# Autodesk Inventor assembly: Battery_Pack
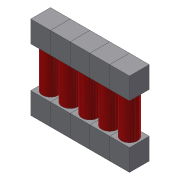
[picture p0: Inventor's stored thumbnail of the model, 180x180]
Saved by Autodesk Inventor 2018 (Build 220112000, 112)
## iProperties
Created: 2019-09-04
Part Number: Battery_Pack
Document SubType Name: Assembly
Designer: Clevo
Author: Clevo
## Documents named in this file (2)
- E:\Hardware_Accelerated_Robot\Hardware\Battery\Battery_Pack.iam
- E:\Hardware_Accelerated_Robot\Hardware\Battery\Battery_Module.iam
## Components (5 placed, 1 different names)
1. Battery_Module:1 [sub-assembly] — Mate:1, Flush:1, Flush:2, Mate:2, Flush:3, Flush:4
2. Battery_Module:2 [sub-assembly] — Mate:1, Flush:1, Flush:2, Mate:4, Flush:7, Flush:8
3. Battery_Module:3 [sub-assembly] — Mate:2, Flush:3, Flush:4, Mate:3, Flush:5, Flush:6
4. Battery_Module:4 [sub-assembly] — Mate:3, Flush:5, Flush:6
5. Battery_Module:5 [sub-assembly] — Mate:4, Flush:7, Flush:8
## Relationships (12: Flush 8, Mate 4)
- Mate:1: Battery_Module:1 ↔ Battery_Module:2
- Flush:1: Battery_Module:1 ↔ Battery_Module:2
- Flush:2: Battery_Module:1 ↔ Battery_Module:2
- Mate:2: Battery_Module:1 ↔ Battery_Module:3
- Flush:3: Battery_Module:1 ↔ Battery_Module:3
- Flush:4: Battery_Module:1 ↔ Battery_Module:3
- Mate:3: Battery_Module:3 ↔ Battery_Module:4
- Flush:5: Battery_Module:3 ↔ Battery_Module:4
- Flush:6: Battery_Module:3 ↔ Battery_Module:4
- Mate:4: Battery_Module:2 ↔ Battery_Module:5
- Flush:7: Battery_Module:2 ↔ Battery_Module:5
- Flush:8: Battery_Module:2 ↔ Battery_Module:5
